# Autodesk Inventor assembly: Assembly_opentrons_microscope_slide_y_base
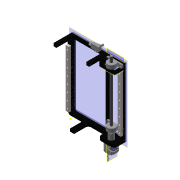
[picture p0: Inventor's stored thumbnail of the model, 180x180]
Saved by Autodesk Inventor 2019.4 (Build 234330000, 330)
## iProperties
Created: 2020-11-05
Part Number: Assembly_opentrons_microscope_slide_y_base
Document SubType Name: Assembly
Designer: diederichbenedict
Author: diederichbenedict
## Documents named in this file (7)
- C:\Users\diederichbenedict\Dropbox\Dokumente\Promotion\PROJECTS\OPENTRONS\INVENTOR\Assembly_opentrons_microscope_slide_y_base.iam
- C:\Users\diederichbenedict\Dropbox\Dokumente\Promotion\PROJECTS\OPENTRONS\INVENTOR\00_NEMA11.iam
- C:\Users\diederichbenedict\Dropbox\Dokumente\Promotion\PROJECTS\OPENTRONS\INVENTOR\Assembly_spindeldrive_350mm_2.iam
- C:\Users\diederichbenedict\Dropbox\Dokumente\Promotion\PROJECTS\OPENTRONS\INVENTOR\02_Opentrons_Microscope_Base_v0.ipt
- C:\Users\diederichbenedict\Dropbox\Dokumente\Promotion\PROJECTS\OPENTRONS\INVENTOR\00_MGN12 LINEAR GUIDE RAIL, CONFIGURABLE.ipt
- C:\Users\diederichbenedict\Dropbox\Dokumente\Promotion\PROJECTS\OPENTRONS\INVENTOR\09_Opentrons_Microscope_Baseplate.ipt
- C:\Users\diederichbenedict\Dropbox\Dokumente\Promotion\PROJECTS\OPENTRONS\INVENTOR\00_Endstop.ipt
## Components (7 placed, 6 different names)
1. 00_MGN12 LINEAR GUIDE RAIL, CONFIGURABLE:1
2. 09_Opentrons_Microscope_Baseplate:1
3. 02_Opentrons_Microscope_Base_v0:1 — Insert:4, Angle:1, Flush:4, Mate:3, Mate:4
4. 00_NEMA11:1 [sub-assembly] — Insert:4, Angle:1
5. Assembly_spindeldrive_350mm_2:1 [sub-assembly]
6. 00_MGN12 LINEAR GUIDE RAIL, CONFIGURABLE:2
7. 00_Endstop:1 — Flush:4, Mate:3, Mate:4
## Relationships (12: Mate 4, Flush 4, Insert 2, Angle 2)
- [Insert] (3 mm): 00_NEMA11:1 ↔ Assembly_spindeldrive_350mm_2:1
- Insert:4: 02_Opentrons_Microscope_Base_v0:1 ↔ 00_NEMA11:1
- Angle:1 (0 deg): 02_Opentrons_Microscope_Base_v0:1 ↔ 00_NEMA11:1
- [Mate]: 00_MGN12 LINEAR GUIDE RAIL, CONFIGURABLE:1 ↔ 02_Opentrons_Microscope_Base_v0:1
- [Flush]: 00_MGN12 LINEAR GUIDE RAIL, CONFIGURABLE:1 ↔ 02_Opentrons_Microscope_Base_v0:1
- [Mate]: 02_Opentrons_Microscope_Base_v0:1 ↔ 00_MGN12 LINEAR GUIDE RAIL, CONFIGURABLE:2
- [Angle] (0 deg): 02_Opentrons_Microscope_Base_v0:1 ↔ 00_MGN12 LINEAR GUIDE RAIL, CONFIGURABLE:2
- [Flush]: 02_Opentrons_Microscope_Base_v0:1 ↔ 00_MGN12 LINEAR GUIDE RAIL, CONFIGURABLE:2
- [Flush]: 09_Opentrons_Microscope_Baseplate:1 ↔ 02_Opentrons_Microscope_Base_v0:1
- Flush:4: 02_Opentrons_Microscope_Base_v0:1 ↔ 00_Endstop:1
- Mate:3: 02_Opentrons_Microscope_Base_v0:1 ↔ 00_Endstop:1
- Mate:4 (5 mm): 02_Opentrons_Microscope_Base_v0:1 ↔ 00_Endstop:1
